# Autodesk Inventor assembly: Arm_Shim
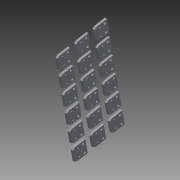
[picture p0: Inventor's stored thumbnail of the model, 180x180]
Saved by Autodesk Inventor 2013 (Build 170138000, 138)
## iProperties
Created: 2014-05-16
Part Number: Arm_Shim
Document SubType Name: Assembly
Designer: andou
Author: andou
## Documents named in this file (2)
- C:\Users\andou\Documents\Inventor\RoboticsProject\project_4\Robot\Arm\Arm_Link_Shim_18.iam
- C:\Users\andou\Documents\Inventor\RoboticsProject\project_4\Robot\Arm\Arm_Link_Shim.ipt
## Components (18 placed, 1 different names)
1. Arm_Link_Shim:1
2. Arm_Link_Shim:2
3. Arm_Link_Shim:3
4. Arm_Link_Shim:4
5. Arm_Link_Shim:5
6. Arm_Link_Shim:6
7. Arm_Link_Shim:7
8. Arm_Link_Shim:8
9. Arm_Link_Shim:9
10. Arm_Link_Shim:10
11. Arm_Link_Shim:11
12. Arm_Link_Shim:12
13. Arm_Link_Shim:13
14. Arm_Link_Shim:14
15. Arm_Link_Shim:15
16. Arm_Link_Shim:16
17. Arm_Link_Shim:17
18. Arm_Link_Shim:18
## Component patterns: (18 elements, first: Arm_Link_Shim:1)
